# Autodesk Inventor assembly: Assembly1
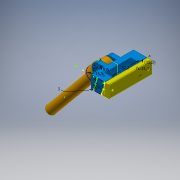
[picture p0: Inventor's stored thumbnail of the model, 180x180]
Saved by Autodesk Inventor 2019 (Build 230136000, 136)
## iProperties
Created: 2021-05-24
Part Number: Assembly1
Material: Genérico
Document SubType Name: Assembly
Designer: Juan M. Casillas
Author: Juan M. Casillas
## Documents named in this file (3)
- K:\3DPrinting\3DModels\clutch\Assembly1.iam
- K:\3DPrinting\3DModels\clutch\pedal_adapter.ipt
- K:\3DPrinting\3DModels\clutch\shaft.ipt
## Components (2 placed, 2 different names)
1. pedal_adapter:1 — Rotational:1
2. shaft:1 — Rotational:1
## Relationships (1: RevoluteJoint 1)
- Rotational:1 [RevoluteJoint]: pedal_adapter:1 ↔ shaft:1
